# Autodesk Inventor assembly: Tool Dock Assembly
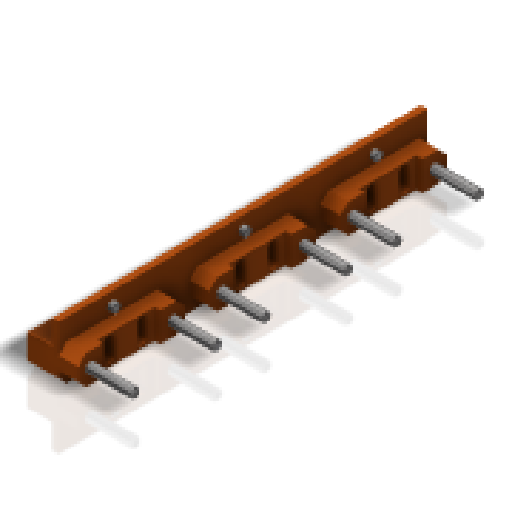
[picture p0: Inventor's stored thumbnail of the model, 512x512]
Saved by Autodesk Inventor 2023.2 (Build 272271000, 271)
## iProperties
Created: 2023-02-06
Part Number: Tool Dock Assembly
Document SubType Name: Assembly
Designer: remop
Author: remop
## Documents named in this file (6)
- C:\Users\remop\OneDrive\Documents\Inventor\3D Printers\LuEVO\Mk5_FullKinematic\Tool Dock Assembly.iam
- C:\Users\remop\OneDrive\Documents\Inventor\3D Printers\LuEVO\Mk5_FullKinematic\Tool Dock Base.ipt
- C:\Users\remop\OneDrive\Documents\Inventor\3D Printers\LuEVO\Mk5_FullKinematic\Tool Dock.ipt
- C:\Users\remop\OneDrive\Documents\Inventor\Content Center Files\R2023\en-US\AS 1420\AS 1420 - 1973 - M3 x 8.ipt
- C:\Users\remop\OneDrive\Documents\Inventor\3D Printers\LuEVO\Mk5_FullKinematic\Tool Dock Bolt.ipt
- C:\Users\remop\OneDrive\Documents\Inventor\Content Center Files\R2023\en-US\AS 1420\AS 1420 - 1973 - M3 x 12.ipt
## Components (16 placed, 5 different names)
1. Tool Dock Base:1 — Flush:1, Mate:1, Flush:2, Mate:2, Mate:3, Insert:1, Insert:2, Insert:3, Rigid:8, Rigid:9, Rigid:10
2. Tool Dock:1 — Flush:1, Mate:1, Flush:2, Flush:3, Flush:4, Mate:4, Mate:5, Rigid:3, Rigid:4
3. Tool Dock:2 — Mate:2, Flush:4, Mate:4, Rigid:5, Rigid:6
4. Tool Dock:3 — Mate:3, Flush:3, Mate:5, Rigid:2, Rigid:7
5. AS 1420 - Metric M3 x 8:1 — Insert:1
6. AS 1420 - Metric M3 x 8:2 — Insert:2
7. AS 1420 - Metric M3 x 8:3 — Insert:3
8. Tool Dock Bolt:1 — Rigid:7
9. Tool Dock Bolt:2 — Rigid:4
10. Tool Dock Bolt:3 — Rigid:5
11. Tool Dock Bolt:4 — Rigid:6
12. Tool Dock Bolt:5 — Rigid:2
13. Tool Dock Bolt:6 — Rigid:3
14. AS 1420 - Metric M3 x 12:1 — Rigid:8
15. AS 1420 - Metric M3 x 12:2 — Rigid:10
16. AS 1420 - Metric M3 x 12:3 — Rigid:9
## Relationships (21: WeldJoint 9, Mate 5, Flush 4, Insert 3)
- Flush:1 (4 mm): Tool Dock Base:1 ↔ Tool Dock:1
- Mate:1: Tool Dock Base:1 ↔ Tool Dock:1
- Flush:2 (80 mm): Tool Dock Base:1 ↔ Tool Dock:1
- Mate:2: Tool Dock Base:1 ↔ Tool Dock:2
- Mate:3: Tool Dock Base:1 ↔ Tool Dock:3
- Flush:3: Tool Dock:1 ↔ Tool Dock:3
- Flush:4: Tool Dock:1 ↔ Tool Dock:2
- Mate:4 (15 mm): Tool Dock:1 ↔ Tool Dock:2
- Mate:5 (15 mm): Tool Dock:1 ↔ Tool Dock:3
- Insert:1: Tool Dock Base:1 ↔ AS 1420 - Metric M3 x 8:1
- Insert:2: Tool Dock Base:1 ↔ AS 1420 - Metric M3 x 8:2
- Insert:3: Tool Dock Base:1 ↔ AS 1420 - Metric M3 x 8:3
- Rigid:2 [WeldJoint]: Tool Dock:3 ↔ Tool Dock Bolt:5
- Rigid:3 [WeldJoint]: Tool Dock:1 ↔ Tool Dock Bolt:6
- Rigid:4 [WeldJoint]: Tool Dock:1 ↔ Tool Dock Bolt:2
- Rigid:5 [WeldJoint]: Tool Dock:2 ↔ Tool Dock Bolt:3
- Rigid:6 [WeldJoint]: Tool Dock:2 ↔ Tool Dock Bolt:4
- Rigid:7 [WeldJoint]: Tool Dock:3 ↔ Tool Dock Bolt:1
- Rigid:8 [WeldJoint] (2 mm): Tool Dock Base:1 ↔ AS 1420 - Metric M3 x 12:1
- Rigid:9 [WeldJoint] (2 mm): Tool Dock Base:1 ↔ AS 1420 - Metric M3 x 12:3
- Rigid:10 [WeldJoint] (2 mm): Tool Dock Base:1 ↔ AS 1420 - Metric M3 x 12:2
